# Autodesk Inventor assembly: De truc Z
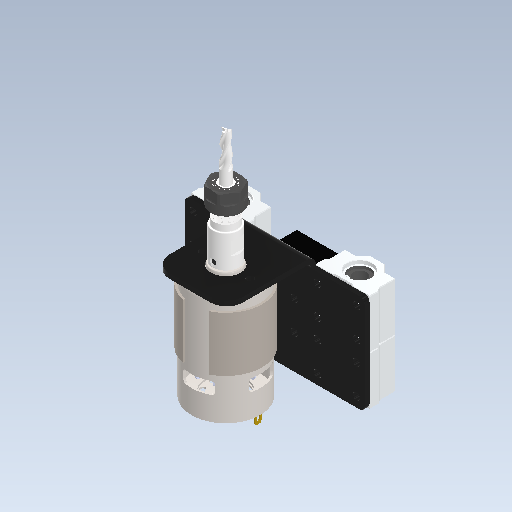
[picture p0: Inventor's stored thumbnail of the model, 512x512]
Saved by Autodesk Inventor 2020 (Build 240168000, 168)
## iProperties
Created: 2021-05-25
Part Number: De truc Z
Document SubType Name: Assembly
Designer: admin
Author: admin
## Documents named in this file (7)
- C:\Users\Admin\Downloads\CNC phay mach\De truc Z.iam
- C:\Users\Admin\Downloads\CNC phay mach\SC8uu.ipt
- C:\Users\Admin\Downloads\CNC phay mach\AoVitmeT8.ipt
- C:\Users\Admin\Downloads\CNC phay mach\De truc Z chan sat.ipt
- C:\Users\Admin\Downloads\CNC phay mach\T8 Nut.ipt
- C:\Users\Admin\Downloads\CNC phay mach\Dong co 775.ipt
- C:\Users\Admin\Downloads\CNC phay mach\Bo collect ER11\C16-ER11-35L 5mm Shank Chuck Collet.iam
## Components (9 placed, 6 different names)
1. SC8uu:1 — Mate:11, Mate:12, Mate:13
2. AoVitmeT8:1 — Mate:23, Mate:24, Mate:25, Mate:32, Mate:33
3. SC8uu:2 — Mate:14, Mate:15, Mate:16
4. SC8uu:3 — Mate:17, Mate:18, Mate:19
5. SC8uu:4 — Mate:20, Mate:21, Mate:22
6. De truc Z chan sat:1 — Mate:11, Mate:12, Mate:13, Mate:14, Mate:15, Mate:16, Mate:17, Mate:18, Mate:19, Mate:20, Mate:21, Mate:22, Mate:23, Mate:24, Mate:25, Mate:34
7. Dong co 775:1 — Mate:35
8. T8 Nut:1 — Mate:32, Mate:33
9. C16-ER11-35L 5mm Shank Chuck Collet:1 [sub-assembly] — Mate:34, Mate:35
## Relationships (21: Mate 21)
- Mate:11: SC8uu:1 ↔ De truc Z chan sat:1
- Mate:12: SC8uu:1 ↔ De truc Z chan sat:1
- Mate:13: SC8uu:1 ↔ De truc Z chan sat:1
- Mate:14: SC8uu:2 ↔ De truc Z chan sat:1
- Mate:15: SC8uu:2 ↔ De truc Z chan sat:1
- Mate:16: SC8uu:2 ↔ De truc Z chan sat:1
- Mate:17: SC8uu:3 ↔ De truc Z chan sat:1
- Mate:18: SC8uu:3 ↔ De truc Z chan sat:1
- Mate:19: SC8uu:3 ↔ De truc Z chan sat:1
- Mate:20: SC8uu:4 ↔ De truc Z chan sat:1
- Mate:21: SC8uu:4 ↔ De truc Z chan sat:1
- Mate:22: SC8uu:4 ↔ De truc Z chan sat:1
- Mate:23: AoVitmeT8:1 ↔ De truc Z chan sat:1
- Mate:24: AoVitmeT8:1 ↔ De truc Z chan sat:1
- Mate:25: AoVitmeT8:1 ↔ De truc Z chan sat:1
- [Mate]: De truc Z chan sat:1 ↔ Dong co 775:1
- [Mate]: De truc Z chan sat:1 ↔ Dong co 775:1
- Mate:32: AoVitmeT8:1 ↔ T8 Nut:1
- Mate:33: AoVitmeT8:1 ↔ T8 Nut:1
- Mate:34 (2 mm): De truc Z chan sat:1 ↔ C16-ER11-35L 5mm Shank Chuck Collet:1
- Mate:35: Dong co 775:1 ↔ C16-ER11-35L 5mm Shank Chuck Collet:1
